# Autodesk Inventor assembly: full_assembly
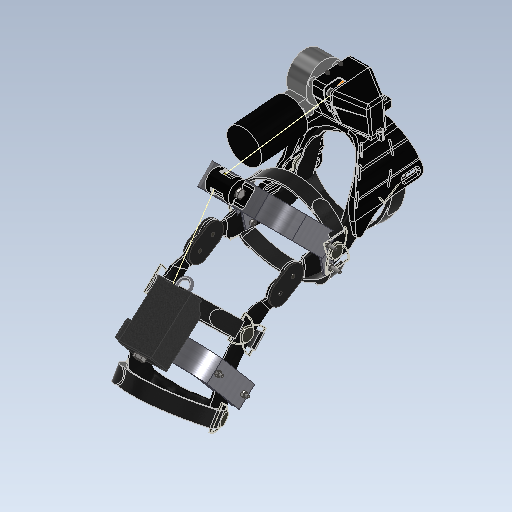
[picture p0: Inventor's stored thumbnail of the model, 512x512]
Saved by Autodesk Inventor 2025.2 (Build 292293000, 293)
## iProperties
Created: 2025-02-17
Part Number: full_assembly
Document SubType Name: Assembly
Designer: email
Author: email
## Documents named in this file (7)
- C:\Users\email\Desktop\Projects\Capstone\4TB6\CAD_Model\thigh_mount_2\full_assembly.iam
- C:\Users\email\Desktop\Projects\Capstone\4TB6\CAD_Model\thigh_mount_2\thighmount_assembly_2.1.iam
- C:\Users\email\Desktop\Projects\Capstone\4TB6\CAD_Model\thigh_mount_2\hinge.ipt
- C:\Users\email\Desktop\Projects\Capstone\4TB6\CAD_Model\thigh_mount_2\rivet.ipt
- C:\Users\email\Desktop\Projects\Capstone\4TB6\CAD_Model\thigh_mount_2\shin_assembly.iam
- C:\Users\email\Desktop\Projects\Capstone\4TB6\CAD_Model\thigh_mount_2\rope.ipt
- C:\Users\email\Desktop\Projects\Capstone\4TB6\CAD_Model\thigh_mount_2\spool_temp.ipt
## Components (12 placed, 6 different names)
1. thighmount_assembly_2.1:1 [sub-assembly] — Mate:1, Mate:5, Mate:9, Mate:10, Mate:12, Mate:18, Flush:5, Angle:1, Mate:22, Mate:23
2. hinge:1 — Mate:3, Mate:4, Mate:5, Flush:1, Flush:2, Mate:20
3. hinge:2 — Mate:7, Mate:8, Mate:9
4. hinge:3 — Mate:16, Mate:17, Mate:18
5. hinge:4 — Mate:12, Mate:14, Mate:15, Flush:3, Flush:4
6. rivet:1 — Mate:1, Mate:3, Flush:1, Mate:7
7. rivet:2 — Mate:4, Flush:2, Mate:8, Mate:19
8. rivet:3 — Mate:10, Mate:14, Flush:3, Mate:16
9. rivet:4 — Mate:15, Flush:4, Mate:17, Mate:21
10. shin_assembly:1 [sub-assembly] — Mate:19, Mate:20, Mate:21, Flush:5, Angle:1, Rotation:1
11. rope:1
12. spool_temp:1 — Mate:22, Mate:23, Rotation:1
## Relationships (26: Mate 19, Flush 5, Angle 1, RelateRotation 1)
- Mate:1: thighmount_assembly_2.1:1 ↔ rivet:1
- Mate:3: hinge:1 ↔ rivet:1
- Mate:4: hinge:1 ↔ rivet:2
- Mate:5: thighmount_assembly_2.1:1 ↔ hinge:1
- Flush:1: hinge:1 ↔ rivet:1
- Flush:2: hinge:1 ↔ rivet:2
- Mate:7: hinge:2 ↔ rivet:1
- Mate:8: hinge:2 ↔ rivet:2
- Mate:9: thighmount_assembly_2.1:1 ↔ hinge:2
- Mate:10: thighmount_assembly_2.1:1 ↔ rivet:3
- Mate:12: thighmount_assembly_2.1:1 ↔ hinge:4
- Mate:14: hinge:4 ↔ rivet:3
- Mate:15: hinge:4 ↔ rivet:4
- Flush:3: hinge:4 ↔ rivet:3
- Flush:4: hinge:4 ↔ rivet:4
- Mate:16: hinge:3 ↔ rivet:3
- Mate:17: hinge:3 ↔ rivet:4
- Mate:18: thighmount_assembly_2.1:1 ↔ hinge:3
- Mate:19: rivet:2 ↔ shin_assembly:1
- Mate:20: hinge:1 ↔ shin_assembly:1
- Mate:21: rivet:4 ↔ shin_assembly:1
- Flush:5: thighmount_assembly_2.1:1 ↔ shin_assembly:1
- Angle:1 (130 deg): thighmount_assembly_2.1:1 ↔ shin_assembly:1
- Mate:22: thighmount_assembly_2.1:1 ↔ spool_temp:1
- Mate:23: thighmount_assembly_2.1:1 ↔ spool_temp:1
- Rotation:1 [RelateRotation] (6 ul): shin_assembly:1 ↔ spool_temp:1
